# Autodesk Inventor assembly: Loop Assembly
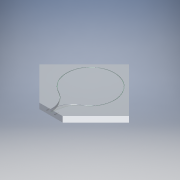
[picture p0: Inventor's stored thumbnail of the model, 180x180]
Saved by Autodesk Inventor 2016 (Build 200138000, 138)
## iProperties
Created: 2015-08-17
Part Number: Loop Assembly
Document SubType Name: Assembly
Designer: Cosmic
Author: Cosmic
## Documents named in this file (4)
- C:\Users\Jonathan\Documents\Projects\loop\scintillatorPanel\loopPanel.iam
- C:\Users\Jonathan\Documents\Projects\loop\scintillatorPanel\loopPanel.ipt
- C:\Users\Jonathan\Documents\Projects\loop\scintillatorPanel\fiberLoop.ipt
- C:\Users\Jonathan\Documents\Projects\loop\scintillatorPanel\Scintillator.xlsx
## Components (2 placed, 2 different names)
1. loopPanel:1 — Mate:1, Mate:2, Flush:1, Mate:3
2. fiberLoop:1 — Mate:1, Mate:2, Flush:1, Mate:3
## Relationships (4: Mate 3, Flush 1)
- Mate:1: loopPanel:1 ↔ fiberLoop:1
- Mate:2: loopPanel:1 ↔ fiberLoop:1
- Flush:1: loopPanel:1 ↔ fiberLoop:1
- Mate:3: loopPanel:1 ↔ fiberLoop:1
## Named parameters: OpticalFiberClearence = 0.15 mm, MPPCClearence = 0.075 mm, FiberSensorClerence = 0.5 mm, OpticalFiberDiameter = 0.8 mm, ScintillatorThickness = 12.7 mm, SmallTrackDiameter = 175 mm, LargeTrackRatio = 3, ScintillatorEdgeClearence = 3 mm, ScintillatorWidth = 146.05 mm, ScintillatorHeight = 146.05 mm, ShallowTrackDepth = 1 mm, MPPCSensorClearence = 1.45 mm, MPPCSensorOffsett = 2.105 mm, MPPCWidth = 5.9 mm, MPPCHeight = 6.55 mm, FiberEdgeOffsett = 5 mm, MPPCDepth = 1 mm, LongFiberAngle = 30 deg, ShortFiberAngle = 78 deg, LoopLargeTrackRatio = 1.2, LoopSmallTrackDiameter = 90 mm, MountingScrewDepth = 4 mm, MountingScrewOffsett = 9 mm, LoopLength = 140 mm, CornerCut = 38.1 mm, FiberSensorClerance = 0.5 mm, DeepTrackDepth = 6.85 mm, OpticalFiberClearance = 0.1 mm, ScintillatorEdgeClearance = 3 mm
